# Autodesk Inventor assembly: Swing-Arm Assembly
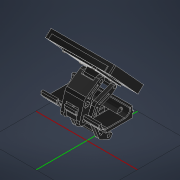
[picture p0: Inventor's stored thumbnail of the model, 180x180]
Saved by Autodesk Inventor 2022.2 (Build 262287010, 287A)
## iProperties
Created: 2022-03-22
Part Number: Swing-Arm Assembly
Document SubType Name: Assembly
Designer: sleib
Author: sleib
## Documents named in this file (12)
- C:\Users\sleib\Projekte\Voron-2\CAD\Inventor\Display Mount\Swing-Arm Assembly.iam
- C:\Users\sleib\Projekte\Voron-2\CAD\Inventor\Display Mount\Skirt Front.ipt
- C:\Users\sleib\Projekte\Voron-2\CAD\Inventor\Display Mount\Swing-Arm C.ipt
- C:\Users\sleib\Projekte\Voron-2\CAD\Inventor\Display Mount\Skirt Mount.ipt
- C:\Users\sleib\Projekte\Voron-2\CAD\Inventor\Display Mount\Swing-Arm A.ipt
- C:\Users\sleib\Projekte\Voron-2\CAD\Inventor\Display Mount\Base-Plate.ipt
- C:\Users\sleib\Projekte\Voron-2\CAD\Inventor\M3 Threaded Insert.ipt
- C:\Users\sleib\Projekte\Voron-2\CAD\Inventor\M3x12 SHCS.ipt
- C:\Users\sleib\Projekte\Voron-2\CAD\Inventor\M3x8 SHCS.ipt
- C:\Users\sleib\Projekte\Voron-2\CAD\Inventor\M3 Hexnut.ipt
- C:\Users\sleib\Projekte\Voron-2\CAD\Inventor\Display Mount\Swing-Arm B.ipt
- C:\Users\sleib\Projekte\Voron-2\CAD\Inventor\Display Mount\Display-Bevel.ipt
## Components (23 placed, 11 different names)
1. Skirt Front:1 — Passend:2, Passend:3, Fluchtend:1, Drehbar:1, Passend:13, Passend:14, Fluchtend:3, Fluchtend:4, Passend:19, Passend:20, Passend:21, Passend:22
2. Skirt Mount:1 — Passend:3, Fluchtend:1, Fluchtend:2, Passend:5, Passend:7, Drehbar:2, Drehbar:3, Passend:17, Passend:18
3. Base-Plate:1 — Passend:11, Passend:12, Drehbar:4, Drehbar:5, Drehbar:6, Passend:31, Passend:32, Passend:33, Passend:34, Passend:35, Passend:36, Passend:37, Passend:42
4. Swing-Arm C:1 — Passend:2, Fluchtend:2, Drehbar:1, Drehbar:6, Passend:23, Passend:24, Passend:25, Passend:26, Winkel:1, Winkel:2
5. Swing-Arm A:1 — Passend:5, Passend:12, Drehbar:3, Drehbar:5
6. Swing-Arm B:1 — Passend:7, Passend:11, Drehbar:2, Drehbar:4
7. M3 Threaded Insert:1 — Passend:13, Fluchtend:3, Passend:16
8. M3 Threaded Insert:2 — Passend:14, Fluchtend:4, Passend:15
9. M3x12 SHCS:1 — Passend:16, Passend:17
10. M3x12 SHCS:2 — Passend:15, Passend:18
11. M3x8 SHCS:1 — Passend:19, Passend:22
12. M3x8 SHCS:2 — Passend:20, Passend:21
13. M3 Hexnut:1 — Passend:23, Passend:26, Winkel:1
14. M3 Hexnut:2 — Passend:24, Passend:25, Winkel:2
15. Display-Bevel:1 — Passend:27, Passend:28, Passend:29, Passend:30, Fluchtend:5, Fluchtend:6, Fluchtend:7, Fluchtend:8, Passend:42
16. M3 Threaded Insert:3 — Passend:27, Fluchtend:8, Passend:39
17. M3 Threaded Insert:4 — Passend:28, Fluchtend:7, Passend:38
18. M3 Threaded Insert:5 — Passend:29, Fluchtend:5, Passend:41
19. M3 Threaded Insert:6 — Passend:30, Fluchtend:6, Passend:40
20. M3x8 SHCS:3 — Passend:31, Passend:39
21. M3x8 SHCS:4 — Passend:33, Passend:36, Passend:40
22. M3x8 SHCS:5 — Passend:34, Passend:35, Passend:38
23. M3x8 SHCS:6 — Passend:32, Passend:37, Passend:41
## Relationships (52: Mate 36, Flush 8, RevoluteJoint 6, Angle 2)
- Passend:2 [Mate]: Skirt Front:1 ↔ Swing-Arm C:1
- Passend:3 [Mate]: Skirt Front:1 ↔ Skirt Mount:1
- Fluchtend:1 [Flush]: Skirt Front:1 ↔ Skirt Mount:1
- Fluchtend:2 [Flush]: Skirt Mount:1 ↔ Swing-Arm C:1
- Passend:5 [Mate]: Skirt Mount:1 ↔ Swing-Arm A:1
- Passend:7 [Mate]: Skirt Mount:1 ↔ Swing-Arm B:1
- Passend:11 [Mate]: Base-Plate:1 ↔ Swing-Arm B:1
- Passend:12 [Mate]: Base-Plate:1 ↔ Swing-Arm A:1
- Drehbar:1 [RevoluteJoint]: Skirt Front:1 ↔ Swing-Arm C:1
- Drehbar:2 [RevoluteJoint]: Skirt Mount:1 ↔ Swing-Arm B:1
- Drehbar:3 [RevoluteJoint]: Skirt Mount:1 ↔ Swing-Arm A:1
- Drehbar:4 [RevoluteJoint]: Base-Plate:1 ↔ Swing-Arm B:1
- Drehbar:5 [RevoluteJoint]: Base-Plate:1 ↔ Swing-Arm A:1
- Drehbar:6 [RevoluteJoint]: Base-Plate:1 ↔ Swing-Arm C:1
- Passend:13 [Mate]: Skirt Front:1 ↔ M3 Threaded Insert:1
- Passend:14 [Mate]: Skirt Front:1 ↔ M3 Threaded Insert:2
- Fluchtend:3 [Flush]: Skirt Front:1 ↔ M3 Threaded Insert:1
- Fluchtend:4 [Flush]: Skirt Front:1 ↔ M3 Threaded Insert:2
- Passend:15 [Mate]: M3 Threaded Insert:2 ↔ M3x12 SHCS:2
- Passend:16 [Mate]: M3 Threaded Insert:1 ↔ M3x12 SHCS:1
- Passend:17 [Mate]: Skirt Mount:1 ↔ M3x12 SHCS:1
- Passend:18 [Mate]: Skirt Mount:1 ↔ M3x12 SHCS:2
- Passend:19 [Mate]: Skirt Front:1 ↔ M3x8 SHCS:1
- Passend:20 [Mate]: Skirt Front:1 ↔ M3x8 SHCS:2
- Passend:21 [Mate]: Skirt Front:1 ↔ M3x8 SHCS:2
- Passend:22 [Mate]: Skirt Front:1 ↔ M3x8 SHCS:1
- Passend:23 [Mate]: Swing-Arm C:1 ↔ M3 Hexnut:1
- Passend:24 [Mate]: Swing-Arm C:1 ↔ M3 Hexnut:2
- Passend:25 [Mate]: Swing-Arm C:1 ↔ M3 Hexnut:2
- Passend:26 [Mate]: Swing-Arm C:1 ↔ M3 Hexnut:1
- Winkel:1 [Angle] (0 deg): Swing-Arm C:1 ↔ M3 Hexnut:1
- Winkel:2 [Angle] (0 deg): Swing-Arm C:1 ↔ M3 Hexnut:2
- Passend:27 [Mate]: Display-Bevel:1 ↔ M3 Threaded Insert:3
- Passend:28 [Mate]: Display-Bevel:1 ↔ M3 Threaded Insert:4
- Passend:29 [Mate]: Display-Bevel:1 ↔ M3 Threaded Insert:5
- Passend:30 [Mate]: Display-Bevel:1 ↔ M3 Threaded Insert:6
- Fluchtend:5 [Flush]: Display-Bevel:1 ↔ M3 Threaded Insert:5
- Fluchtend:6 [Flush]: Display-Bevel:1 ↔ M3 Threaded Insert:6
- Fluchtend:7 [Flush]: Display-Bevel:1 ↔ M3 Threaded Insert:4
- Fluchtend:8 [Flush]: Display-Bevel:1 ↔ M3 Threaded Insert:3
- Passend:31 [Mate]: Base-Plate:1 ↔ M3x8 SHCS:3
- Passend:32 [Mate]: Base-Plate:1 ↔ M3x8 SHCS:6
- Passend:33 [Mate]: Base-Plate:1 ↔ M3x8 SHCS:4
- Passend:34 [Mate]: Base-Plate:1 ↔ M3x8 SHCS:5
- Passend:35 [Mate]: Base-Plate:1 ↔ M3x8 SHCS:5
- Passend:36 [Mate]: Base-Plate:1 ↔ M3x8 SHCS:4
- Passend:37 [Mate]: Base-Plate:1 ↔ M3x8 SHCS:6
- Passend:38 [Mate]: M3 Threaded Insert:4 ↔ M3x8 SHCS:5
- Passend:39 [Mate]: M3 Threaded Insert:3 ↔ M3x8 SHCS:3
- Passend:40 [Mate]: M3 Threaded Insert:6 ↔ M3x8 SHCS:4
- Passend:41 [Mate]: M3 Threaded Insert:5 ↔ M3x8 SHCS:6
- Passend:42 [Mate]: Base-Plate:1 ↔ Display-Bevel:1
